# Autodesk Inventor assembly: Remote_Station
(part 2 of 2)
- [Insert]: Internal Tooth Lock Washer - Type A (Inch) No. 4. Carbon Steel:25 ↔ Hexagon Socket Button Head Cap Screw - Inch 4 - 40 - 3/4:25
- [Insert]: Plain Washer (Inch) No. 4 - narrow - Type B:25 ↔ Internal Tooth Lock Washer - Type A (Inch) No. 4. Carbon Steel:25
- [Insert]: Internal Tooth Lock Washer - Type A (Inch) No. 4. Carbon Steel:26 ↔ Hexagon Socket Button Head Cap Screw - Inch 4 - 40 - 3/4:26
- [Insert]: Plain Washer (Inch) No. 4 - narrow - Type B:26 ↔ Internal Tooth Lock Washer - Type A (Inch) No. 4. Carbon Steel:26
- [Insert]: KWBH0001:7 ↔ Plain Washer (Inch) No. 4 - narrow - Type B:25
- [Insert]: KWBH0001:7 ↔ Plain Washer (Inch) No. 4 - narrow - Type B:26
- [Insert]: Internal Tooth Lock Washer - Type A (Inch) No. 4. Carbon Steel:27 ↔ Hexagon Socket Button Head Cap Screw - Inch 4 - 40 - 3/4:27
- [Insert]: Plain Washer (Inch) No. 4 - narrow - Type B:27 ↔ Internal Tooth Lock Washer - Type A (Inch) No. 4. Carbon Steel:27
- [Insert]: Internal Tooth Lock Washer - Type A (Inch) No. 4. Carbon Steel:28 ↔ Hexagon Socket Button Head Cap Screw - Inch 4 - 40 - 3/4:28
- [Insert]: Plain Washer (Inch) No. 4 - narrow - Type B:28 ↔ Internal Tooth Lock Washer - Type A (Inch) No. 4. Carbon Steel:28
- [Insert]: KWBH0001:8 ↔ Microswitch_Bracket:8
- [Flush]: KWBH0001:8 ↔ Microswitch_Bracket:8
- [Insert]: Internal Tooth Lock Washer - Type A (Inch) No. 4. Carbon Steel:29 ↔ Hexagon Socket Button Head Cap Screw - Inch 4 - 40 - 3/4:29
- [Insert]: Plain Washer (Inch) No. 4 - narrow - Type B:29 ↔ Internal Tooth Lock Washer - Type A (Inch) No. 4. Carbon Steel:29
- [Insert]: Internal Tooth Lock Washer - Type A (Inch) No. 4. Carbon Steel:30 ↔ Hexagon Socket Button Head Cap Screw - Inch 4 - 40 - 3/4:30
- [Insert]: Plain Washer (Inch) No. 4 - narrow - Type B:30 ↔ Internal Tooth Lock Washer - Type A (Inch) No. 4. Carbon Steel:30
- [Insert]: KWBH0001:8 ↔ Plain Washer (Inch) No. 4 - narrow - Type B:29
- [Insert]: KWBH0001:8 ↔ Plain Washer (Inch) No. 4 - narrow - Type B:30
- [Insert]: Internal Tooth Lock Washer - Type A (Inch) No. 4. Carbon Steel:31 ↔ Hexagon Socket Button Head Cap Screw - Inch 4 - 40 - 3/4:31
- [Insert]: Plain Washer (Inch) No. 4 - narrow - Type B:31 ↔ Internal Tooth Lock Washer - Type A (Inch) No. 4. Carbon Steel:31
- [Insert]: Internal Tooth Lock Washer - Type A (Inch) No. 4. Carbon Steel:32 ↔ Hexagon Socket Button Head Cap Screw - Inch 4 - 40 - 3/4:32
- [Insert]: Plain Washer (Inch) No. 4 - narrow - Type B:32 ↔ Internal Tooth Lock Washer - Type A (Inch) No. 4. Carbon Steel:32
- [Insert]: KWBH0001:9 ↔ Microswitch_Bracket:9
- [Flush]: KWBH0001:9 ↔ Microswitch_Bracket:9
- [Insert]: Internal Tooth Lock Washer - Type A (Inch) No. 4. Carbon Steel:33 ↔ Hexagon Socket Button Head Cap Screw - Inch 4 - 40 - 3/4:33
- [Insert]: Plain Washer (Inch) No. 4 - narrow - Type B:33 ↔ Internal Tooth Lock Washer - Type A (Inch) No. 4. Carbon Steel:33
- [Insert]: Internal Tooth Lock Washer - Type A (Inch) No. 4. Carbon Steel:34 ↔ Hexagon Socket Button Head Cap Screw - Inch 4 - 40 - 3/4:34
- [Insert]: Plain Washer (Inch) No. 4 - narrow - Type B:34 ↔ Internal Tooth Lock Washer - Type A (Inch) No. 4. Carbon Steel:34
- [Insert]: KWBH0001:9 ↔ Plain Washer (Inch) No. 4 - narrow - Type B:33
- [Insert]: KWBH0001:9 ↔ Plain Washer (Inch) No. 4 - narrow - Type B:34
- [Insert]: Internal Tooth Lock Washer - Type A (Inch) No. 4. Carbon Steel:35 ↔ Hexagon Socket Button Head Cap Screw - Inch 4 - 40 - 3/4:35
- [Insert]: Plain Washer (Inch) No. 4 - narrow - Type B:35 ↔ Internal Tooth Lock Washer - Type A (Inch) No. 4. Carbon Steel:35
- [Insert]: Internal Tooth Lock Washer - Type A (Inch) No. 4. Carbon Steel:36 ↔ Hexagon Socket Button Head Cap Screw - Inch 4 - 40 - 3/4:36
- [Insert]: Plain Washer (Inch) No. 4 - narrow - Type B:36 ↔ Internal Tooth Lock Washer - Type A (Inch) No. 4. Carbon Steel:36
- [Insert]: KWBH0001:10 ↔ Microswitch_Bracket:10
- [Flush]: KWBH0001:10 ↔ Microswitch_Bracket:10
- [Insert]: Internal Tooth Lock Washer - Type A (Inch) No. 4. Carbon Steel:37 ↔ Hexagon Socket Button Head Cap Screw - Inch 4 - 40 - 3/4:37
- [Insert]: Plain Washer (Inch) No. 4 - narrow - Type B:37 ↔ Internal Tooth Lock Washer - Type A (Inch) No. 4. Carbon Steel:37
- [Insert]: Internal Tooth Lock Washer - Type A (Inch) No. 4. Carbon Steel:38 ↔ Hexagon Socket Button Head Cap Screw - Inch 4 - 40 - 3/4:38
- [Insert]: Plain Washer (Inch) No. 4 - narrow - Type B:38 ↔ Internal Tooth Lock Washer - Type A (Inch) No. 4. Carbon Steel:38
- [Insert]: KWBH0001:10 ↔ Plain Washer (Inch) No. 4 - narrow - Type B:37
- [Insert]: KWBH0001:10 ↔ Plain Washer (Inch) No. 4 - narrow - Type B:38
- [Insert]: Internal Tooth Lock Washer - Type A (Inch) No. 4. Carbon Steel:39 ↔ Hexagon Socket Button Head Cap Screw - Inch 4 - 40 - 3/4:39
- [Insert]: Plain Washer (Inch) No. 4 - narrow - Type B:39 ↔ Internal Tooth Lock Washer - Type A (Inch) No. 4. Carbon Steel:39
- [Insert]: Internal Tooth Lock Washer - Type A (Inch) No. 4. Carbon Steel:40 ↔ Hexagon Socket Button Head Cap Screw - Inch 4 - 40 - 3/4:40
- [Insert]: Plain Washer (Inch) No. 4 - narrow - Type B:40 ↔ Internal Tooth Lock Washer - Type A (Inch) No. 4. Carbon Steel:40
- Mate:18: SCESCE-20N2010LP:1 ↔ Microswitch_Bracket:2
- Mate:19: SCESCE-20N2010LP:1 ↔ Microswitch_Bracket:6
- Mate:20: SCESCE-20N2010LP:1 ↔ Microswitch_Bracket:7
- Mate:21: SCESCE-20N2010LP:1 ↔ Microswitch_Bracket:8
- Mate:22: SCESCE-20N2010LP:1 ↔ Microswitch_Bracket:3
- Mate:23: SCESCE-20N2010LP:1 ↔ Microswitch_Bracket:9
- Mate:24: SCESCE-20N2010LP:1 ↔ Microswitch_Bracket:4
- Mate:25: SCESCE-20N2010LP:1 ↔ Microswitch_Bracket:10
- Mate:26: SCESCE-20N2010LP:1 ↔ Microswitch_Bracket:5
- Mate:27: SCESCE-20N2010LP:1 ↔ Microswitch_Bracket:6
- Mate:28: SCESCE-20N2010LP:1 ↔ Microswitch_Bracket:7
- Mate:29: SCESCE-20N2010LP:1 ↔ Microswitch_Bracket:2
- Mate:30: SCESCE-20N2010LP:1 ↔ Microswitch_Bracket:3
- Mate:31: SCESCE-20N2010LP:1 ↔ Microswitch_Bracket:8
- Mate:32: SCESCE-20N2010LP:1 ↔ Microswitch_Bracket:9
- Mate:33: SCESCE-20N2010LP:1 ↔ Microswitch_Bracket:4
- Mate:34: SCESCE-20N2010LP:1 ↔ Microswitch_Bracket:5
- Mate:35: SCESCE-20N2010LP:1 ↔ Microswitch_Bracket:10
- Flush:12: Microswitch_Bracket:1 ↔ Microswitch_Bracket:6
- Flush:13: Microswitch_Bracket:2 ↔ Microswitch_Bracket:7
- Flush:14: Microswitch_Bracket:3 ↔ Microswitch_Bracket:8
- Flush:15: Microswitch_Bracket:4 ↔ Microswitch_Bracket:9
- Insert:248: SCESCE-20N2010LP:1 ↔ Plain Washer (Inch) No. 4 - narrow - Type B:24
- Insert:249: SCESCE-20N2010LP:1 ↔ Plain Washer (Inch) No. 4 - narrow - Type B:23
- Insert:250: SCESCE-20N2010LP:1 ↔ Plain Washer (Inch) No. 4 - narrow - Type B:28
- Insert:251: SCESCE-20N2010LP:1 ↔ Plain Washer (Inch) No. 4 - narrow - Type B:27
- Insert:252: SCESCE-20N2010LP:1 ↔ Plain Washer (Inch) No. 4 - narrow - Type B:8
- Insert:253: SCESCE-20N2010LP:1 ↔ Plain Washer (Inch) No. 4 - narrow - Type B:32
- Insert:254: SCESCE-20N2010LP:1 ↔ Plain Washer (Inch) No. 4 - narrow - Type B:31
- Insert:255: SCESCE-20N2010LP:1 ↔ Plain Washer (Inch) No. 4 - narrow - Type B:36
- Insert:256: SCESCE-20N2010LP:1 ↔ Plain Washer (Inch) No. 4 - narrow - Type B:12
- Insert:257: SCESCE-20N2010LP:1 ↔ Plain Washer (Inch) No. 4 - narrow - Type B:7
- Insert:258: SCESCE-20N2010LP:1 ↔ Plain Washer (Inch) No. 4 - narrow - Type B:11
- Insert:259: SCESCE-20N2010LP:1 ↔ Plain Washer (Inch) No. 4 - narrow - Type B:35
- Insert:260: SCESCE-20N2010LP:1 ↔ Plain Washer (Inch) No. 4 - narrow - Type B:16
- Insert:261: SCESCE-20N2010LP:1 ↔ Plain Washer (Inch) No. 4 - narrow - Type B:15
- Insert:262: SCESCE-20N2010LP:1 ↔ Plain Washer (Inch) No. 4 - narrow - Type B:40
- Insert:263: SCESCE-20N2010LP:1 ↔ Plain Washer (Inch) No. 4 - narrow - Type B:39
- Insert:264: SCESCE-20N2010LP:1 ↔ Plain Washer (Inch) No. 4 - narrow - Type B:19
- Insert:265: SCESCE-20N2010LP:1 ↔ Plain Washer (Inch) No. 4 - narrow - Type B:20
- Mate:36: Deck_Bushing:3 ↔ Fender:6
- Mate:37: Deck_Bushing:10 ↔ Fender:7
- Mate:38: Deck_Bushing:1 ↔ Fender:8
- Mate:39: Deck_Bushing:6 ↔ Fender:2
- Mate:40: Deck_Bushing:2 ↔ Fender:3
- Mate:41: Deck_Bushing:7 ↔ Fender:4
- Mate:42: Deck_Bushing:8 ↔ Fender:9
- Mate:43: Deck_Bushing:4 ↔ Fender:5
- Mate:44: Deck_Bushing:5 ↔ Fender:10
- Flush:16: Fender:1 ↔ Fender:7
- Flush:17: Fender:2 ↔ Fender:7
- Flush:18: Fender:2 ↔ Fender:4
- Flush:19: Fender:4 ↔ Fender:5
- Flush:20: Fender:5 ↔ Fender:10
- Flush:21: Fender:9 ↔ Fender:10
- Flush:22: Fender:3 ↔ Fender:9
- Flush:23: Fender:3 ↔ Fender:8
- Flush:24: Fender:6 ↔ Fender:8
- Insert:266: 9414K360:1 ↔ 9414K930:1
- Insert:267: SCESCE-20N2010LP:1 ↔ 9414K930:1
- Mate:45: Cap_Mount:2 ↔ 3.5F_Cap:1
- Mate:46: Cap_Mount:1 ↔ 3.5F_Cap:1
- Insert:268: SCESCE-20N2010LP:1 ↔ Cap_Mount:1
- Insert:269: SCESCE-20N2010LP:1 ↔ Cap_Mount:2
- [Insert]: Hexagon Socket Head Cap Screw - Inch 10-32 UNF - 0.5:6 ↔ Internal Tooth Lock Washer - Type A (Inch) No. 12. Carbon Steel:31
- [Insert]: Plain Washer (Inch) No. 12 - narrow - Type B:31 ↔ Internal Tooth Lock Washer - Type A (Inch) No. 12. Carbon Steel:31
- [Insert]: Hexagon Socket Head Cap Screw - Inch 10-32 UNF - 0.5:4 ↔ Internal Tooth Lock Washer - Type A (Inch) No. 12. Carbon Steel:32
- [Insert]: Plain Washer (Inch) No. 12 - narrow - Type B:32 ↔ Internal Tooth Lock Washer - Type A (Inch) No. 12. Carbon Steel:32
- [Insert]: Hexagon Socket Head Cap Screw - Inch 10-32 UNF - 0.5:3 ↔ Internal Tooth Lock Washer - Type A (Inch) No. 12. Carbon Steel:33
- [Insert]: Plain Washer (Inch) No. 12 - narrow - Type B:33 ↔ Internal Tooth Lock Washer - Type A (Inch) No. 12. Carbon Steel:33
- [Insert]: Hexagon Socket Head Cap Screw - Inch 10-32 UNF - 0.5:5 ↔ Internal Tooth Lock Washer - Type A (Inch) No. 12. Carbon Steel:34
- [Insert]: Plain Washer (Inch) No. 12 - narrow - Type B:34 ↔ Internal Tooth Lock Washer - Type A (Inch) No. 12. Carbon Steel:34
- Insert:278: Cap_Mount:2 ↔ Plain Washer (Inch) No. 12 - narrow - Type B:31
- Insert:279: Cap_Mount:2 ↔ Plain Washer (Inch) No. 12 - narrow - Type B:34
- Insert:280: Cap_Mount:1 ↔ Plain Washer (Inch) No. 12 - narrow - Type B:33
- Insert:281: Cap_Mount:1 ↔ Plain Washer (Inch) No. 12 - narrow - Type B:32
- [Insert]: Plain Washer (Inch) No. 12 - narrow - Type B:35 ↔ Internal Tooth Lock Washer - Type A (Inch) No. 12. Carbon Steel:35
- [Insert]: Plain Washer (Inch) No. 12 - narrow - Type B:36 ↔ Internal Tooth Lock Washer - Type A (Inch) No. 12. Carbon Steel:36
- [Insert]: Plain Washer (Inch) No. 12 - narrow - Type B:37 ↔ Internal Tooth Lock Washer - Type A (Inch) No. 12. Carbon Steel:37
- [Insert]: Plain Washer (Inch) No. 12 - narrow - Type B:38 ↔ Internal Tooth Lock Washer - Type A (Inch) No. 12. Carbon Steel:38
- Insert:286: SCESCE-20N2010LP:1 ↔ Plain Washer (Inch) No. 12 - narrow - Type B:35
- Insert:287: SCESCE-20N2010LP:1 ↔ Plain Washer (Inch) No. 12 - narrow - Type B:37
- Insert:288: SCESCE-20N2010LP:1 ↔ Plain Washer (Inch) No. 12 - narrow - Type B:38
- Insert:289: SCESCE-20N2010LP:1 ↔ Plain Washer (Inch) No. 12 - narrow - Type B:36
- Insert:290: Internal Tooth Lock Washer - Type A (Inch) No. 12. Carbon Steel:36 ↔ Hex Machine Screw Nut - Inch 10 - 32:1
- Insert:291: Internal Tooth Lock Washer - Type A (Inch) No. 12. Carbon Steel:38 ↔ Hex Machine Screw Nut - Inch 10 - 32:2
- Insert:292: Internal Tooth Lock Washer - Type A (Inch) No. 12. Carbon Steel:35 ↔ Hex Machine Screw Nut - Inch 10 - 32:3
- Insert:293: Internal Tooth Lock Washer - Type A (Inch) No. 12. Carbon Steel:37 ↔ Hex Machine Screw Nut - Inch 10 - 32:4
- Flush:25 (2.54 mm): Cap_Mount:2 ↔ 3.5F_Cap:1
- Insert:294: SCESCE-20N2010LP:1 ↔ Horn:1
- Mate:47: SCESCE-20N2010LP:1 ↔ Horn:1
- Insert:295: Plain Washer (Metric) 8 N:1 ↔ Hex Bolt - Metric M8 x 1.25 x 30:1
- Insert:296: Plain Washer (Metric) 8 N:2 ↔ Hex Bolt - Metric M8 x 1.25 x 30:2
- Insert:297: Plain Washer (Metric) 8 N:3 ↔ Hex Bolt - Metric M8 x 1.25 x 30:3
- Insert:298: Hex Nut Metric M8 x 1.25:2 ↔ Helical Spring Lock Washers 0.375:1
- Insert:299: Hex Nut Metric M8 x 1.25:1 ↔ Helical Spring Lock Washers 0.375:2
- Insert:300: Hex Nut Metric M8 x 1.25:3 ↔ Helical Spring Lock Washers 0.375:3
- Insert:301: Horn:1 ↔ Plain Washer (Metric) 8 N:2
- Insert:302: Horn:1 ↔ Plain Washer (Metric) 8 N:1
- Insert:303: Horn:1 ↔ Plain Washer (Metric) 8 N:3
- Insert:304: SCESCE-20N2010LP:1 ↔ Helical Spring Lock Washers 0.375:1
- Insert:305: SCESCE-20N2010LP:1 ↔ Helical Spring Lock Washers 0.375:2
- Insert:306: SCESCE-20N2010LP:1 ↔ Helical Spring Lock Washers 0.375:3
- Insert:307: SCESCE-20N2010LP:1 ↔ Barrel_Jack:1
- Mate:48: SCESCE-20N2010LP:1 ↔ Barrel_Jack:1
- Insert:308: SCESCE-20N2010LP:1 ↔ Norgren-R07-100-RGEA+18-025-003+18-013-212:1
- Tangent:1: SCESCE-20N2010LP:1 ↔ Norgren-R07-100-RGEA+18-025-003+18-013-212:1
- [Insert]: Hexagon Socket Head Cap Screw - Inch 10-32 UNF - 0.5:2 ↔ Internal Tooth Lock Washer - Type A (Inch) No. 12. Carbon Steel:39
- [Insert]: Plain Washer (Inch) No. 12 - narrow - Type B:39 ↔ Internal Tooth Lock Washer - Type A (Inch) No. 12. Carbon Steel:39
- [Insert]: Plain Washer (Inch) No. 12 - narrow - Type B:40 ↔ Internal Tooth Lock Washer - Type A (Inch) No. 12. Carbon Steel:40
- [Insert]: Internal Tooth Lock Washer - Type A (Inch) No. 12. Carbon Steel:40 ↔ Hex Machine Screw Nut - Inch 10 - 32:5
- [Insert]: Hexagon Socket Head Cap Screw - Inch 10-32 UNF - 0.5:1 ↔ Internal Tooth Lock Washer - Type A (Inch) No. 12. Carbon Steel:41
- [Insert]: Plain Washer (Inch) No. 12 - narrow - Type B:41 ↔ Internal Tooth Lock Washer - Type A (Inch) No. 12. Carbon Steel:41
- [Insert]: Plain Washer (Inch) No. 12 - narrow - Type B:42 ↔ Internal Tooth Lock Washer - Type A (Inch) No. 12. Carbon Steel:42
- [Insert]: Internal Tooth Lock Washer - Type A (Inch) No. 12. Carbon Steel:42 ↔ Hex Machine Screw Nut - Inch 10 - 32:6
- Insert:317: Norgren-R07-100-RGEA+18-025-003+18-013-212:1 ↔ Plain Washer (Inch) No. 12 - narrow - Type B:41
- Insert:318: Norgren-R07-100-RGEA+18-025-003+18-013-212:1 ↔ Plain Washer (Inch) No. 12 - narrow - Type B:39
- Insert:319: SCESCE-20N2010LP:1 ↔ Plain Washer (Inch) No. 12 - narrow - Type B:42
- Insert:320: SCESCE-20N2010LP:1 ↔ Plain Washer (Inch) No. 12 - narrow - Type B:40
- [Insert]: 9414K360:2 ↔ 9414K930:2
- Insert:322: SCESCE-20N2010LP:1 ↔ 9414K930:2
## Named parameters: d27_d25 = 0 mm, d28_d26 = 0 mm, d29_d25 = 0 mm, d30_d26 = 0 mm, d31_d25 = 0 mm, d32_d26 = 0 mm, d33_d25 = 0 mm, d34_d26 = 0 mm, d35_d25 = 0 mm, d36_d26 = 0 mm, d43_d25 = 0 mm, d44_d26 = 0 mm, d45_d25 = 0 mm, d46_d26 = 0 mm, d47_d25 = 0 mm, d48_d26 = 0 mm, d49_d25 = 0 mm, d50_d26 = 0 mm, d51_d25 = 0 mm, d52_d26 = 0 mm, d53_d25 = 0 mm, d54_d26 = 0 mm, d55_d25 = 0 mm, d56_d26 = 0 mm, d57_d25 = 0 mm, d58_d26 = 0 mm, d59_d25 = 0 mm, d60_d26 = 0 mm, d61_d25 = 0 mm, d62_d26 = 0 mm, d63_d25 = 0 mm, d64_d26 = 0 mm, d65_d25 = 0 mm, d66_d26 = 0 mm, d67_d25 = 0 mm, d68_d26 = 0 mm, d69_d25 = 0 mm, d70_d26 = 0 mm, d71_d25 = 0 mm, d72_d26 = 0 mm, d73_d25 = 0 mm, d74_d26 = 0 mm, d75_d25 = 0 mm, d76_d26 = 0 mm, d77_d25 = 0 mm, d78_d26 = 0 mm, d79_d25 = 0 mm, d80_d26 = 0 mm, d81_d25 = 0 mm, d82_d26 = 0 mm, d105_d25 = 0 mm, d106_d26 = 0 mm, d107_d25 = 0 mm, d108_d26 = 0 mm, d111_d25 = 0 mm, d112_d26 = 0 mm, d113_d25 = 0 mm, d114_d26 = 0 mm, d167_d165 = 0 mm, d168_d166 = 0 mm, d177_d165 = 0 mm, d178_d166 = 0 mm, d179_d165 = 0 mm, d180_d166 = 0 mm, d183_d169 = 0 mm, d184_d170 = 0 mm, d185_d177_d165 = 0 mm, d186_d178_d166 = 0 mm, d187_d179_d165 = 0 mm, d188_d180_d166 = 0 mm, d189_d163 = 0 mm, d190_d164 = 0 mm, d191_d165 = 0 mm, d192_d166 = 0 mm, d193_d167_d165 = 0 mm, d194_d168_d166 = 0 mm, d195_d169 = 0 mm, d196_d170 = 0 mm, d197_d177_d165 = 0 mm, d198_d178_d166 = 0 mm, d199_d179_d165 = 0 mm, d200_d180_d166 = 0 mm, d201_d163 = 0 mm, d202_d164 = 0 mm, d203_d165 = 0 mm, d204_d166 = 0 mm, d205_d167_d165 = 0 mm, d206_d168_d166 = 0 mm, d207_d169 = 0 mm, d208_d170 = 0 mm, d209_d177_d165 = 0 mm, d210_d178_d166 = 0 mm, d211_d179_d165 = 0 mm, d212_d180_d166 = 0 mm, d213_d163 = 0 mm, d214_d164 = 0 mm, d215_d165 = 0 mm, d216_d166 = 0 mm, d217_d167_d165 = 0 mm, d218_d168_d166 = 0 mm, d219_d169 = 0 mm, d220_d170 = 0 mm, d221_d177_d165 = 0 mm, d222_d178_d166 = 0 mm, d223_d179_d165 = 0 mm, d224_d180_d166 = 0 mm, d225_d163 = 0 mm, d226_d164 = 0 mm, d227_d165 = 0 mm, d228_d166 = 0 mm, d229_d167_d165 = 0 mm, d230_d168_d166 = 0 mm, d231_d169 = 0 mm, d232_d170 = 0 mm, d233_d177_d165 = 0 mm, d234_d178_d166 = 0 mm, d235_d179_d165 = 0 mm, d236_d180_d166 = 0 mm, d237_d163 = 0 mm, d238_d164 = 0 mm, d239_d165 = 0 mm, d240_d166 = 0 mm, d241_d167_d165 = 0 mm, d242_d168_d166 = 0 mm, d243_d169 = 0 mm, d244_d170 = 0 mm, d245_d177_d165 = 0 mm, d246_d178_d166 = 0 mm, d247_d179_d165 = 0 mm, d248_d180_d166 = 0 mm, d249_d163 = 0 mm, d250_d164 = 0 mm, d251_d165 = 0 mm, d252_d166 = 0 mm, d253_d167_d165 = 0 mm, d254_d168_d166 = 0 mm, d255_d169 = 0 mm, d256_d170 = 0 mm, d257_d177_d165 = 0 mm, d258_d178_d166 = 0 mm, d259_d179_d165 = 0 mm, d260_d180_d166 = 0 mm, d261_d163 = 0 mm, d262_d164 = 0 mm, d263_d165 = 0 mm, d264_d166 = 0 mm, d265_d167_d165 = 0 mm, d266_d168_d166 = 0 mm, d267_d169 = 0 mm, d268_d170 = 0 mm, d269_d177_d165 = 0 mm, d270_d178_d166 = 0 mm, d271_d179_d165 = 0 mm, d272_d180_d166 = 0 mm, d273_d163 = 0 mm, d274_d164 = 0 mm, d275_d165 = 0 mm, d276_d166 = 0 mm, d277_d167_d165 = 0 mm, d278_d168_d166 = 0 mm, d279_d169 = 0 mm, d280_d170 = 0 mm, d281_d177_d165 = 0 mm, d282_d178_d166 = 0 mm, d283_d179_d165 = 0 mm, d284_d180_d166 = 0 mm, d285_d163 = 0 mm, d286_d164 = 0 mm, d287_d165 = 0 mm, d288_d166 = 0 mm, d289_d167_d165 = 0 mm, d290_d168_d166 = 0 mm, d357_d25 = 0 mm, d358_d26 = 0 mm, d359_d25 = 0 mm, d360_d26 = 0 mm, d361_d25 = 0 mm, d362_d26 = 0 mm, d363_d25 = 0 mm, d364_d26 = 0 mm, d369_d358_d26 = 0 mm, d370_d358_d26 = 0 mm, d371_d358_d26 = 0 mm, d372_d358_d26 = 0 mm, d400_d361_d25 = 0 mm, d401_d362_d26 = 0 mm, d402_d372_d358_d26 = 0 mm, d403_d378 = 0 mm, d404_d361_d25 = 0 mm, d405_d362_d26 = 0 mm, d406_d372_d358_d26 = 0 mm, d407_d378 = 0 mm, d412_d349 = 0 mm
